# Autodesk Inventor assembly: ShooterPrototype-ver1-1111-2019
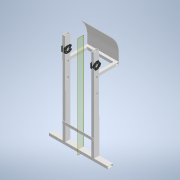
[picture p0: Inventor's stored thumbnail of the model, 180x180]
Saved by Autodesk Inventor 2021 (Build 250183000, 183)
## iProperties
Created: 2020-01-17
Part Number: ShooterPrototype-ver1-1111-2019
Document SubType Name: Assembly
Designer: JMHal
Author: JMHal
## Documents named in this file (9)
- C:\Users\con_c_000\Documents\GitHub\RoboticsCad1111\PHRC CADD\2020 Infinite Recharge\Shooting\Assemblies\ShooterPrototype-ver2-1111-2019.iam
- C:\Users\con_c_000\Documents\GitHub\RoboticsCad1111\PHRC CADD\2020 Infinite Recharge\Shooting\Parts\12in 2x1 Aluminum Block-ver1-1111-2019.ipt
- C:\Users\con_c_000\Documents\GitHub\RoboticsCad1111\PHRC CADD\2020 Infinite Recharge\Shooting\Parts\16in 2x1 Aluminum Block-ver1-1111-2019.ipt
- C:\Users\con_c_000\Documents\GitHub\RoboticsCad1111\PHRC CADD\2020 Infinite Recharge\Shooting\Parts\12in Aluminum Plate-ver-1-1111-2019.ipt
- C:\Users\con_c_000\Documents\GitHub\RoboticsCad1111\PHRC CADD\2020 Infinite Recharge\Shooting\Parts\VersaBlock-ver1-1111-2019.ipt
- C:\Users\con_c_000\Documents\GitHub\RoboticsCad1111\PHRC CADD\Resources\VEXpro Resources\Bearings\0.5inHexFlangedBearing(1.125inx0.313in)-1111-2016.ipt
- C:\Users\con_c_000\Documents\GitHub\RoboticsCad1111\PHRC CADD\2020 Infinite Recharge\Shooting\Parts\ShooterBracket.ver1-1111-2020.ipt
- C:\Users\con_c_000\Documents\GitHub\RoboticsCad1111\PHRC CADD\2020 Infinite Recharge\Shooting\Parts\ShooterBracketHorizontal.ver1-1111-2020.ipt
- C:\Users\con_c_000\Documents\GitHub\RoboticsCad1111\PHRC CADD\2020 Infinite Recharge\Shooting\Parts\Hood.ver1-1111-2020.ipt
## Components (16 placed, 8 different names)
1. 12in 2x1 Aluminum Block-ver1-1111-2019:1 — Mate:22, Flush:5, Flush:6, Flush:7
2. 12in Aluminum Plate-ver-1-1111-2019:1 — Mate:12, Mate:13, Flush:2
3. 16in 2x1 Aluminum Block-ver1-1111-2019:3 — Mate:12, Mate:13, Mate:15, Cylindrical:2, Mate:16, Angle:1, Cylindrical:5, Mate:18, Angle:3, Flush:4, Flush:7, Symmetry:1, Flush:16, Mate:29
4. 16in 2x1 Aluminum Block-ver1-1111-2019:4 — Cylindrical:3, Mate:17, Cylindrical:6, Mate:19, Angle:4, Flush:2, Flush:4, Mate:22, Flush:5, Flush:6, Symmetry:1, Flush:15, Mate:28
5. VersaBlock-ver1-1111-2019:1 — Mate:15, Angle:1, Rotational:1
6. 0.5inHexFlangedBearing(1.125inx0.313in)-1111-2016:1 — Cylindrical:2, Mate:16, Rotational:1
7. 0.5inHexFlangedBearing(1.125inx0.313in)-1111-2016:2 — Cylindrical:3, Mate:17, Rotational:2
8. VersaBlock-ver1-1111-2019:2 — Rotational:2
9. 0.5inHexFlangedBearing(1.125inx0.313in)-1111-2016:3 — Cylindrical:5, Mate:18, Rotational:3
10. VersaBlock-ver1-1111-2019:3 — Rotational:3, Angle:3
11. VersaBlock-ver1-1111-2019:4 — Rotational:4, Angle:4
12. 0.5inHexFlangedBearing(1.125inx0.313in)-1111-2016:4 — Cylindrical:6, Mate:19, Rotational:4
13. ShooterBracket.ver1-1111-2020:1 — Flush:10, Flush:15, Mate:28
14. ShooterBracket.ver1-1111-2020:2 — Flush:10, Mate:26, Flush:12, Flush:16, Mate:29, Flush:17
15. ShooterBracketHorizontal.ver1-1111-2020:1 — Mate:26, Flush:12, Mate:27, Flush:14, Flush:17, Flush:18
16. Hood.ver1-1111-2020:1 — Mate:27, Flush:14, Flush:18
## Relationships (36: Mate 12, Flush 12, CylindricalJoint 4, RevoluteJoint 4, Angle 3, Symmetry 1)
- Mate:12: 12in Aluminum Plate-ver-1-1111-2019:1 ↔ 16in 2x1 Aluminum Block-ver1-1111-2019:3
- Mate:13: 12in Aluminum Plate-ver-1-1111-2019:1 ↔ 16in 2x1 Aluminum Block-ver1-1111-2019:3
- Mate:15: 16in 2x1 Aluminum Block-ver1-1111-2019:3 ↔ VersaBlock-ver1-1111-2019:1
- Cylindrical:2: 16in 2x1 Aluminum Block-ver1-1111-2019:3 ↔ 0.5inHexFlangedBearing(1.125inx0.313in)-1111-2016:1
- Mate:16: 16in 2x1 Aluminum Block-ver1-1111-2019:3 ↔ 0.5inHexFlangedBearing(1.125inx0.313in)-1111-2016:1
- Cylindrical:3: 16in 2x1 Aluminum Block-ver1-1111-2019:4 ↔ 0.5inHexFlangedBearing(1.125inx0.313in)-1111-2016:2
- Mate:17: 16in 2x1 Aluminum Block-ver1-1111-2019:4 ↔ 0.5inHexFlangedBearing(1.125inx0.313in)-1111-2016:2
- Angle:1 (0 deg): 16in 2x1 Aluminum Block-ver1-1111-2019:3 ↔ VersaBlock-ver1-1111-2019:1
- Rotational:1 [RevoluteJoint]: VersaBlock-ver1-1111-2019:1 ↔ 0.5inHexFlangedBearing(1.125inx0.313in)-1111-2016:1
- Rotational:2 [RevoluteJoint]: 0.5inHexFlangedBearing(1.125inx0.313in)-1111-2016:2 ↔ VersaBlock-ver1-1111-2019:2
- Cylindrical:5: 16in 2x1 Aluminum Block-ver1-1111-2019:3 ↔ 0.5inHexFlangedBearing(1.125inx0.313in)-1111-2016:3
- Mate:18: 16in 2x1 Aluminum Block-ver1-1111-2019:3 ↔ 0.5inHexFlangedBearing(1.125inx0.313in)-1111-2016:3
- Rotational:3 [RevoluteJoint]: 0.5inHexFlangedBearing(1.125inx0.313in)-1111-2016:3 ↔ VersaBlock-ver1-1111-2019:3
- Angle:3 (0 deg): 16in 2x1 Aluminum Block-ver1-1111-2019:3 ↔ VersaBlock-ver1-1111-2019:3
- Cylindrical:6: 16in 2x1 Aluminum Block-ver1-1111-2019:4 ↔ 0.5inHexFlangedBearing(1.125inx0.313in)-1111-2016:4
- Mate:19: 16in 2x1 Aluminum Block-ver1-1111-2019:4 ↔ 0.5inHexFlangedBearing(1.125inx0.313in)-1111-2016:4
- Rotational:4 [RevoluteJoint]: VersaBlock-ver1-1111-2019:4 ↔ 0.5inHexFlangedBearing(1.125inx0.313in)-1111-2016:4
- Angle:4 (0 deg): 16in 2x1 Aluminum Block-ver1-1111-2019:4 ↔ VersaBlock-ver1-1111-2019:4
- Flush:2: 12in Aluminum Plate-ver-1-1111-2019:1 ↔ 16in 2x1 Aluminum Block-ver1-1111-2019:4
- Flush:4: 16in 2x1 Aluminum Block-ver1-1111-2019:3 ↔ 16in 2x1 Aluminum Block-ver1-1111-2019:4
- Mate:22: 12in 2x1 Aluminum Block-ver1-1111-2019:1 ↔ 16in 2x1 Aluminum Block-ver1-1111-2019:4
- Flush:5: 12in 2x1 Aluminum Block-ver1-1111-2019:1 ↔ 16in 2x1 Aluminum Block-ver1-1111-2019:4
- Flush:6 (-133.35 mm): 12in 2x1 Aluminum Block-ver1-1111-2019:1 ↔ 16in 2x1 Aluminum Block-ver1-1111-2019:4
- Flush:7: 12in 2x1 Aluminum Block-ver1-1111-2019:1 ↔ 16in 2x1 Aluminum Block-ver1-1111-2019:3
- Flush:10: ShooterBracket.ver1-1111-2020:1 ↔ ShooterBracket.ver1-1111-2020:2
- Mate:26: ShooterBracket.ver1-1111-2020:2 ↔ ShooterBracketHorizontal.ver1-1111-2020:1
- Flush:12: ShooterBracket.ver1-1111-2020:2 ↔ ShooterBracketHorizontal.ver1-1111-2020:1
- Mate:27: ShooterBracketHorizontal.ver1-1111-2020:1 ↔ Hood.ver1-1111-2020:1
- Flush:14: ShooterBracketHorizontal.ver1-1111-2020:1 ↔ Hood.ver1-1111-2020:1
- Symmetry:1: 16in 2x1 Aluminum Block-ver1-1111-2019:3 ↔ 16in 2x1 Aluminum Block-ver1-1111-2019:4
- Flush:15: 16in 2x1 Aluminum Block-ver1-1111-2019:4 ↔ ShooterBracket.ver1-1111-2020:1
- Mate:28: 16in 2x1 Aluminum Block-ver1-1111-2019:4 ↔ ShooterBracket.ver1-1111-2020:1
- Flush:16: 16in 2x1 Aluminum Block-ver1-1111-2019:3 ↔ ShooterBracket.ver1-1111-2020:2
- Mate:29: 16in 2x1 Aluminum Block-ver1-1111-2019:3 ↔ ShooterBracket.ver1-1111-2020:2
- Flush:17: ShooterBracket.ver1-1111-2020:2 ↔ ShooterBracketHorizontal.ver1-1111-2020:1
- Flush:18: ShooterBracketHorizontal.ver1-1111-2020:1 ↔ Hood.ver1-1111-2020:1
